# Autodesk Inventor assembly: 0005-00-03 Y axis
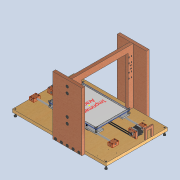
[picture p0: Inventor's stored thumbnail of the model, 180x180]
Saved by Autodesk Inventor 2020 (Build 240168000, 168)
## iProperties
Created: 2020-12-18
Part Number: 0005-00-03 Y axis
Document SubType Name: Assembly
Designer: Iulian Bors
Mass: 17144.8 g
Surface Area: 27601.7 cm^2
Volume: 16303.9 cm^3
Density: 1.05157 g/cm^3
Author: Iulian Bors
Subject: 10-03
## Documents named in this file (29)
- Z:\I.A.B\Proiecte\0005 I.A.B 3d 2.0 Imprimanta aracet\10 Mecanic\0005-10-03 Y axis.iam
- Z:\I.A.B\Proiecte\0005 I.A.B 3d 2.0 Imprimanta aracet\10 Mecanic\Foaie A4.ipt
- Z:\I.A.B\Proiecte\0005 I.A.B 3d 2.0 Imprimanta aracet\10 Mecanic\0005-10-1001 NEMA17 - Motor de passo.ipt
- Z:\I.A.B\Proiecte\0005 I.A.B 3d 2.0 Imprimanta aracet\10 Mecanic\0005-10-013 Bed.ipt
- Z:\I.A.B\Proiecte\0005 I.A.B 3d 2.0 Imprimanta aracet\10 Mecanic\0005-10-1008 Bara rectificata.ipt
- Z:\I.A.B\Proiecte\0005 I.A.B 3d 2.0 Imprimanta aracet\10 Mecanic\0005-10-014 Suport Bed.ipt
- Z:\I.A.B\Proiecte\0005 I.A.B 3d 2.0 Imprimanta aracet\10 Mecanic\0005-10-1009 LM10uu.ipt
- Z:\I.A.B\Proiecte\0005 I.A.B 3d 2.0 Imprimanta aracet\10 Mecanic\0005-10-015 suport tija.ipt
- Z:\I.A.B\Proiecte\0005 I.A.B 3d 2.0 Imprimanta aracet\10 Mecanic\0005-10-1010 GT2 Timing Pulley 20 Tooth.ipt
- Z:\I.A.B\Proiecte\0005 I.A.B 3d 2.0 Imprimanta aracet\10 Mecanic\0005-10-1011 16T W6 B3 Without T_Shrinkwrap_1.ipt
- Z:\I.A.B\Proiecte\0005 I.A.B 3d 2.0 Imprimanta aracet\10 Mecanic\0005-10-019 intinzator y.ipt
- Z:\I.A.B\Proiecte\0005 I.A.B 3d 2.0 Imprimanta aracet\10 Mecanic\0005-10-1016 curea Y.ipt
- Z:\I.A.B\Proiecte\0005 I.A.B 3d 2.0 Imprimanta aracet\10 Mecanic\0005-10-020 suport motor y.ipt
- Z:\I.A.B\Proiecte\0005 I.A.B 3d 2.0 Imprimanta aracet\10 Mecanic\0005-10-025 Activator senzor Y.ipt
- Z:\I.A.B\Proiecte\0005 I.A.B 3d 2.0 Imprimanta aracet\10 Mecanic\0005-10-1035.ipt
- Z:\I.A.B\Proiecte\0005 I.A.B 3d 2.0 Imprimanta aracet\10 Mecanic\0005-10-1036 DIN 125 - A 5.3.ipt
- Z:\I.A.B\Proiecte\0005 I.A.B 3d 2.0 Imprimanta aracet\10 Mecanic\0005-10-1037 DIN 315 - M4.ipt
- Z:\I.A.B\Proiecte\0005 I.A.B 3d 2.0 Imprimanta aracet\10 Mecanic\0005-10-1033 DIN 914 - M5 x 10.ipt
- Z:\I.A.B\Proiecte\0005 I.A.B 3d 2.0 Imprimanta aracet\10 Mecanic\0005-10-1032.ipt
- Z:\I.A.B\Proiecte\0005 I.A.B 3d 2.0 Imprimanta aracet\10 Mecanic\0005-10-1020 ISO 7089 - 3 - 140 HV(1).ipt
- Z:\I.A.B\Proiecte\0005 I.A.B 3d 2.0 Imprimanta aracet\10 Mecanic\Surub M4 saiba piulita 60mm.iam
- Z:\I.A.B\Proiecte\0005 I.A.B 3d 2.0 Imprimanta aracet\10 Mecanic\Surub M4 saiba piulita 45mm.iam
- Z:\I.A.B\Proiecte\0005 I.A.B 3d 2.0 Imprimanta aracet\10 Mecanic\0005-10-1040 Coil.iam
- Z:\I.A.B\Proiecte\0005 I.A.B 3d 2.0 Imprimanta aracet\10 Mecanic\Colier.ipt
- Z:\I.A.B\Proiecte\0005 I.A.B 3d 2.0 Imprimanta aracet\10 Mecanic\0005-10-01 Cadru_Shrinkwrap_1.ipt
- Z:\I.A.B\Proiecte\0005 I.A.B 3d 2.0 Imprimanta aracet\10 Mecanic\0005-10-1049 DIN 7991 - M4x40.ipt
- Z:\I.A.B\Proiecte\0005 I.A.B 3d 2.0 Imprimanta aracet\10 Mecanic\0005-10-1027 ISO 7050 - ST 4.2 x 32 - C - Z.ipt
- Z:\I.A.B\Proiecte\0005 I.A.B 3d 2.0 Imprimanta aracet\10 Mecanic\0005-10-1045ISO 7050 - ST 3.5 x 22 - C - Z.ipt
- Z:\I.A.B\Proiecte\0005 I.A.B 3d 2.0 Imprimanta aracet\10 Mecanic\0005-10-1051 DIN 933 - M5  x 40.ipt
## Components (80 placed, 28 different names)
1. Foaie A4.ipt:1 — Flush:29, Flush:30, Mate:47
2. 0005-10-014 Suport Bed.ipt:2 — Flush:28, Tangent:11, Tangent:12, Flush:29, Flush:30, Mate:46, Flush:32, Flush:33, Mate:48, Mate:125, Flush:67, Insert:30, Insert:31, Insert:32, Insert:33, Flush:71, Mate:132, Mate:135, Mate:136, Angle:19, Angle:20
3. 0005-10-013 Bed.ipt:7 — Mate:47, Flush:32, Flush:33, Mate:48, Insert:26, Insert:27, Insert:28, Insert:29
4. 0005-10-1001 NEMA17 - Motor de passo.ipt:8 — Mate:102, Flush:55, Flush:58
5. 0005-10-1010 GT2 Timing Pulley 20 Tooth.ipt:9 — Mate:94, Mate:95, Flush:51
6. 0005-10-1011 16T W6 B3 Without T_Shrinkwrap_1.ipt:10 — Flush:51
7. 0005-10-019 intinzator y.ipt:11 — Angle:17, Mate:128, Mate:129, Insert:22, Insert:46, Insert:47
8. 0005-10-1016 curea Y.ipt:12 — Mate:94, Mate:95, Angle:17
9. 0005-10-020 suport motor y.ipt:13 — Mate:102, Flush:55, Insert:42, Insert:43, Insert:44, Insert:45, Mate:149
10. 0005-10-025 Activator senzor Y.ipt:14 — Mate:125, Flush:67, Flush:68, Insert:52, Insert:53
11. 0005-10-01 Cadru_Shrinkwrap_1.ipt:15 — Mate:127, Flush:70, Mate:129, Angle:18, Mate:130, Insert:60, Insert:61, Insert:62, Mate:149
12. DIN 933 - M5  x 40.ipt:16 — Insert:22, Insert:23, Insert:25
13. 0005-10-1035.ipt:17 — Insert:23, Insert:24
14. 0005-10-1036 DIN 125 - A 5.3.ipt:18 — Insert:24
15. 0005-10-1036 DIN 125 - A 5.3.ipt:19 — Insert:25
16. 0005-10-1037 DIN 315 - M4.ipt:20 — Insert:26
17. 0005-10-1037 DIN 315 - M4.ipt:21 — Insert:27
18. 0005-10-1037 DIN 315 - M4.ipt:22 — Insert:28
19. 0005-10-1037 DIN 315 - M4.ipt:23 — Insert:29
20. 0005-10-1049 DIN 7991 - M4x40.ipt:24 — Insert:30, Mate:137, Mate:138
21. 0005-10-1049 DIN 7991 - M4x40.ipt:25 — Insert:31, Mate:131
22. 0005-10-1049 DIN 7991 - M4x40.ipt:26 — Insert:32, Mate:133, Mate:134
23. 0005-10-1049 DIN 7991 - M4x40.ipt:27 — Insert:33, Mate:139, Mate:140
24. 0005-10-1033 DIN 914 - M5 x 10.ipt:28 — Insert:35
25. 0005-10-1033 DIN 914 - M5 x 10.ipt:29 — Insert:54
26. 0005-10-1033 DIN 914 - M5 x 10.ipt:30 — Insert:37
27. 0005-10-1032.ipt:31
28. 0005-10-1020 ISO 7089 - 3 - 140 HV(1).ipt:32 — Insert:45
29. 0005-10-1032.ipt:33
30. 0005-10-1020 ISO 7089 - 3 - 140 HV(1).ipt:34 — Insert:44
31. 0005-10-1032.ipt:35
32. 0005-10-1020 ISO 7089 - 3 - 140 HV(1).ipt:36 — Insert:43
33. 0005-10-1032.ipt:37
34. 0005-10-1020 ISO 7089 - 3 - 140 HV(1).ipt:38 — Insert:42
35. Surub M4 saiba piulita 60mm.iam:39 [sub-assembly] — Insert:46
36. Surub M4 saiba piulita 60mm.iam:40 [sub-assembly] — Insert:47, Mate:128
37. 0005-10-1045ISO 7050 - ST 3.5 x 22 - C - Z.ipt:41 — Insert:52
38. 0005-10-1045ISO 7050 - ST 3.5 x 22 - C - Z.ipt:42 — Insert:53
39. 0005-10-1033 DIN 914 - M5 x 10.ipt:49 — Insert:55
40. 0005-10-1040 Coil.iam:66 [sub-assembly] — Mate:131, Flush:71
41. 0005-10-1040 Coil.iam:67 [sub-assembly] — Mate:132, Mate:133, Mate:134
42. 0005-10-1040 Coil.iam:68 [sub-assembly] — Mate:136, Mate:137, Mate:138
43. 0005-10-1040 Coil.iam:69 [sub-assembly] — Mate:135, Mate:139, Mate:140
44. Colier.ipt:70 — Mate:145, Flush:79, Angle:20, Flush:81, Flush:83
45. Colier.ipt:71 — Mate:144, Flush:77, Flush:78
46. Colier.ipt:72 — Mate:141, Flush:72, Angle:19, Flush:73
47. Colier.ipt:73 — Mate:143, Flush:75, Flush:76, Flush:78
48. Colier.ipt:74 — Mate:142, Flush:73, Flush:74, Flush:76
49. Colier.ipt:75 — Mate:146, Flush:80, Flush:81, Flush:85
50. Colier.ipt:76 — Mate:148, Flush:84, Flush:85
51. Colier.ipt:77 — Mate:147, Flush:82, Flush:83
52. 0005-10-1027 ISO 7050 - ST 4.2 x 32 - C - Z.ipt:78 — Insert:60
53. 0005-10-1027 ISO 7050 - ST 4.2 x 32 - C - Z.ipt:79 — Insert:61
54. 0005-10-1027 ISO 7050 - ST 4.2 x 32 - C - Z.ipt:80 — Insert:62
55. 0005-10-1009 LM10uu.ipt:3 — Flush:28, Tangent:11, Tangent:12, Mate:147, Flush:82, Mate:148, Flush:84
56. 0005-10-1009 LM10uu.ipt:4 — Mate:44, Mate:63, Mate:141, Flush:72, Mate:142, Flush:74
57. 0005-10-1009 LM10uu.ipt:5 — Flush:68, Mate:145, Flush:79, Mate:146, Flush:80
58. 0005-10-1009 LM10uu.ipt:6 — Mate:65, Mate:143, Flush:75, Mate:144, Flush:77
59. 0005-10-015 suport tija.ipt:43 — Mate:63, Flush:37, Mate:126, Mate:127, Flush:70, Insert:35, Angle:18, Insert:56
60. 0005-10-1008 Bara rectificata.ipt:44 — Mate:44, Flush:37, Mate:126, Flush:69
61. 0005-10-015 suport tija.ipt:45 — Mate:65, Flush:69, Insert:37, Mate:130, Insert:58
62. 0005-10-015 suport tija.ipt:46 — Insert:55, Insert:57
63. 0005-10-1008 Bara rectificata.ipt:47
64. 0005-10-015 suport tija.ipt:48 — Insert:54, Insert:59
65. Surub M4 saiba piulita 45mm.iam:50 [sub-assembly] — Insert:56
66. Surub M4 saiba piulita 45mm.iam:51 [sub-assembly]
67. Surub M4 saiba piulita 45mm.iam:52 [sub-assembly]
68. Surub M4 saiba piulita 45mm.iam:53 [sub-assembly]
69. Surub M4 saiba piulita 45mm.iam:54 [sub-assembly] — Insert:57
70. Surub M4 saiba piulita 45mm.iam:55 [sub-assembly]
71. Surub M4 saiba piulita 45mm.iam:56 [sub-assembly]
72. Surub M4 saiba piulita 45mm.iam:57 [sub-assembly]
73. Surub M4 saiba piulita 45mm.iam:58 [sub-assembly] — Insert:58
74. Surub M4 saiba piulita 45mm.iam:59 [sub-assembly]
75. Surub M4 saiba piulita 45mm.iam:60 [sub-assembly]
76. Surub M4 saiba piulita 45mm.iam:61 [sub-assembly]
77. Surub M4 saiba piulita 45mm.iam:62 [sub-assembly] — Insert:59
78. Surub M4 saiba piulita 45mm.iam:63 [sub-assembly]
79. Surub M4 saiba piulita 45mm.iam:64 [sub-assembly]
80. Surub M4 saiba piulita 45mm.iam:65 [sub-assembly]
## Component patterns: (4 elements, first: 0005-10-1009 LM10uu.ipt:3), (2 elements, first: 0005-10-015 suport tija.ipt:43 + 0005-10-1008 Bara rectificata.ipt:44 + 0005-10-015 suport tija.ipt:45), (4 elements, first: Surub M4 saiba piulita 45mm.iam:50), (4 elements, first: Surub M4 saiba piulita 45mm.iam:54), (4 elements, first: Surub M4 saiba piulita 45mm.iam:58), (4 elements, first: Surub M4 saiba piulita 45mm.iam:62)
## Relationships (106: Mate 36, Insert 36, Flush 28, Angle 4, Tangent 2)
- Flush:28 (75 mm): 0005-10-014 Suport Bed.ipt:2 ↔ 0005-10-1009 LM10uu.ipt:3
- Tangent:11: 0005-10-014 Suport Bed.ipt:2 ↔ 0005-10-1009 LM10uu.ipt:3
- Tangent:12 (-30 mm): 0005-10-014 Suport Bed.ipt:2 ↔ 0005-10-1009 LM10uu.ipt:3
- Mate:44: 0005-10-1009 LM10uu.ipt:4 ↔ 0005-10-1008 Bara rectificata.ipt:44
- Flush:29 (10 mm): Foaie A4.ipt:1 ↔ 0005-10-014 Suport Bed.ipt:2
- Flush:30 (12.5 mm): Foaie A4.ipt:1 ↔ 0005-10-014 Suport Bed.ipt:2
- Mate:46 (18 mm): 0005-10-014 Suport Bed.ipt:2
- Mate:47: Foaie A4.ipt:1 ↔ 0005-10-013 Bed.ipt:7
- Flush:32: 0005-10-014 Suport Bed.ipt:2 ↔ 0005-10-013 Bed.ipt:7
- Flush:33: 0005-10-014 Suport Bed.ipt:2 ↔ 0005-10-013 Bed.ipt:7
- Mate:48 (20 mm): 0005-10-014 Suport Bed.ipt:2 ↔ 0005-10-013 Bed.ipt:7
- Mate:63: 0005-10-1009 LM10uu.ipt:4 ↔ 0005-10-015 suport tija.ipt:43
- Flush:37: 0005-10-015 suport tija.ipt:43 ↔ 0005-10-1008 Bara rectificata.ipt:44
- Mate:65: 0005-10-1009 LM10uu.ipt:6 ↔ 0005-10-015 suport tija.ipt:45
- [Insert] (-13 mm): 0005-10-1001 NEMA17 - Motor de passo.ipt:8 ↔ 0005-10-1010 GT2 Timing Pulley 20 Tooth.ipt:9
- [Mate]: 0005-10-1011 16T W6 B3 Without T_Shrinkwrap_1.ipt:10 ↔ 0005-10-019 intinzator y.ipt:11
- [Mate] (1 mm): 0005-10-1011 16T W6 B3 Without T_Shrinkwrap_1.ipt:10 ↔ 0005-10-019 intinzator y.ipt:11
- Mate:94: 0005-10-1010 GT2 Timing Pulley 20 Tooth.ipt:9 ↔ 0005-10-1016 curea Y.ipt:12
- Mate:95: 0005-10-1010 GT2 Timing Pulley 20 Tooth.ipt:9 ↔ 0005-10-1016 curea Y.ipt:12
- Flush:51: 0005-10-1010 GT2 Timing Pulley 20 Tooth.ipt:9 ↔ 0005-10-1011 16T W6 B3 Without T_Shrinkwrap_1.ipt:10
- Angle:17 (0 deg): 0005-10-019 intinzator y.ipt:11 ↔ 0005-10-1016 curea Y.ipt:12
- Mate:102: 0005-10-1001 NEMA17 - Motor de passo.ipt:8 ↔ 0005-10-020 suport motor y.ipt:13
- Flush:55: 0005-10-1001 NEMA17 - Motor de passo.ipt:8 ↔ 0005-10-020 suport motor y.ipt:13
- Flush:58 (-322.09 mm): 0005-10-1001 NEMA17 - Motor de passo.ipt:8
- Mate:125: 0005-10-014 Suport Bed.ipt:2 ↔ 0005-10-025 Activator senzor Y.ipt:14
- Flush:67: 0005-10-014 Suport Bed.ipt:2 ↔ 0005-10-025 Activator senzor Y.ipt:14
- Flush:68 (-5 mm): 0005-10-025 Activator senzor Y.ipt:14 ↔ 0005-10-1009 LM10uu.ipt:5
- Mate:126: 0005-10-015 suport tija.ipt:43 ↔ 0005-10-1008 Bara rectificata.ipt:44
- Flush:69: 0005-10-1008 Bara rectificata.ipt:44 ↔ 0005-10-015 suport tija.ipt:45
- Mate:127: 0005-10-01 Cadru_Shrinkwrap_1.ipt:15 ↔ 0005-10-015 suport tija.ipt:43
- Flush:70 (5 mm): 0005-10-01 Cadru_Shrinkwrap_1.ipt:15 ↔ 0005-10-015 suport tija.ipt:43
- Mate:128: 0005-10-019 intinzator y.ipt:11 ↔ Surub M4 saiba piulita 60mm.iam:40
- Mate:129: 0005-10-019 intinzator y.ipt:11 ↔ 0005-10-01 Cadru_Shrinkwrap_1.ipt:15
- Insert:22 (1.2 mm): 0005-10-019 intinzator y.ipt:11 ↔ DIN 933 - M5  x 40.ipt:16
- Insert:23 (5 mm): DIN 933 - M5  x 40.ipt:16 ↔ 0005-10-1035.ipt:17
- Insert:24: 0005-10-1035.ipt:17 ↔ 0005-10-1036 DIN 125 - A 5.3.ipt:18
- Insert:25: DIN 933 - M5  x 40.ipt:16 ↔ 0005-10-1036 DIN 125 - A 5.3.ipt:19
- Insert:26: 0005-10-013 Bed.ipt:7 ↔ 0005-10-1037 DIN 315 - M4.ipt:20
- Insert:27: 0005-10-013 Bed.ipt:7 ↔ 0005-10-1037 DIN 315 - M4.ipt:21
- Insert:28: 0005-10-013 Bed.ipt:7 ↔ 0005-10-1037 DIN 315 - M4.ipt:22
- Insert:29: 0005-10-013 Bed.ipt:7 ↔ 0005-10-1037 DIN 315 - M4.ipt:23
- Insert:30: 0005-10-014 Suport Bed.ipt:2 ↔ 0005-10-1049 DIN 7991 - M4x40.ipt:24
- Insert:31: 0005-10-014 Suport Bed.ipt:2 ↔ 0005-10-1049 DIN 7991 - M4x40.ipt:25
- Insert:32: 0005-10-014 Suport Bed.ipt:2 ↔ 0005-10-1049 DIN 7991 - M4x40.ipt:26
- Insert:33: 0005-10-014 Suport Bed.ipt:2 ↔ 0005-10-1049 DIN 7991 - M4x40.ipt:27
- Insert:35: 0005-10-1033 DIN 914 - M5 x 10.ipt:28 ↔ 0005-10-015 suport tija.ipt:43
- Insert:37: 0005-10-1033 DIN 914 - M5 x 10.ipt:30 ↔ 0005-10-015 suport tija.ipt:45
- [Insert]: 0005-10-1032.ipt:31 ↔ 0005-10-1020 ISO 7089 - 3 - 140 HV(1).ipt:32
- [Insert]: 0005-10-1032.ipt:33 ↔ 0005-10-1020 ISO 7089 - 3 - 140 HV(1).ipt:34
- [Insert]: 0005-10-1032.ipt:35 ↔ 0005-10-1020 ISO 7089 - 3 - 140 HV(1).ipt:36
- [Insert]: 0005-10-1032.ipt:37 ↔ 0005-10-1020 ISO 7089 - 3 - 140 HV(1).ipt:38
- Insert:42: 0005-10-020 suport motor y.ipt:13 ↔ 0005-10-1020 ISO 7089 - 3 - 140 HV(1).ipt:38
- Insert:43: 0005-10-020 suport motor y.ipt:13 ↔ 0005-10-1020 ISO 7089 - 3 - 140 HV(1).ipt:36
- Insert:44: 0005-10-020 suport motor y.ipt:13 ↔ 0005-10-1020 ISO 7089 - 3 - 140 HV(1).ipt:34
- Insert:45: 0005-10-020 suport motor y.ipt:13 ↔ 0005-10-1020 ISO 7089 - 3 - 140 HV(1).ipt:32
- Insert:46: 0005-10-019 intinzator y.ipt:11 ↔ Surub M4 saiba piulita 60mm.iam:39
- Insert:47: 0005-10-019 intinzator y.ipt:11 ↔ Surub M4 saiba piulita 60mm.iam:40
- Insert:52: 0005-10-025 Activator senzor Y.ipt:14 ↔ 0005-10-1045ISO 7050 - ST 3.5 x 22 - C - Z.ipt:41
- Insert:53: 0005-10-025 Activator senzor Y.ipt:14 ↔ 0005-10-1045ISO 7050 - ST 3.5 x 22 - C - Z.ipt:42
- Angle:18 (0 deg): 0005-10-01 Cadru_Shrinkwrap_1.ipt:15 ↔ 0005-10-015 suport tija.ipt:43
- Mate:130: 0005-10-01 Cadru_Shrinkwrap_1.ipt:15 ↔ 0005-10-015 suport tija.ipt:45
- Insert:54: 0005-10-1033 DIN 914 - M5 x 10.ipt:29 ↔ 0005-10-015 suport tija.ipt:48
- Insert:55: 0005-10-1033 DIN 914 - M5 x 10.ipt:49 ↔ 0005-10-015 suport tija.ipt:46
- Insert:56: 0005-10-015 suport tija.ipt:43 ↔ Surub M4 saiba piulita 45mm.iam:50
- Insert:57: 0005-10-015 suport tija.ipt:46 ↔ Surub M4 saiba piulita 45mm.iam:54
- Insert:58: 0005-10-015 suport tija.ipt:45 ↔ Surub M4 saiba piulita 45mm.iam:58
- Insert:59: 0005-10-015 suport tija.ipt:48 ↔ Surub M4 saiba piulita 45mm.iam:62
- Mate:131: 0005-10-1049 DIN 7991 - M4x40.ipt:25 ↔ 0005-10-1040 Coil.iam:66
- Flush:71: 0005-10-014 Suport Bed.ipt:2 ↔ 0005-10-1040 Coil.iam:66
- Mate:132: 0005-10-014 Suport Bed.ipt:2 ↔ 0005-10-1040 Coil.iam:67
- Mate:133: 0005-10-1049 DIN 7991 - M4x40.ipt:26 ↔ 0005-10-1040 Coil.iam:67
- Mate:134: 0005-10-1049 DIN 7991 - M4x40.ipt:26 ↔ 0005-10-1040 Coil.iam:67
- Mate:135: 0005-10-014 Suport Bed.ipt:2 ↔ 0005-10-1040 Coil.iam:69
- Mate:136: 0005-10-014 Suport Bed.ipt:2 ↔ 0005-10-1040 Coil.iam:68
- Mate:137: 0005-10-1049 DIN 7991 - M4x40.ipt:24 ↔ 0005-10-1040 Coil.iam:68
- Mate:138: 0005-10-1049 DIN 7991 - M4x40.ipt:24 ↔ 0005-10-1040 Coil.iam:68
- Mate:139: 0005-10-1049 DIN 7991 - M4x40.ipt:27 ↔ 0005-10-1040 Coil.iam:69
- Mate:140: 0005-10-1049 DIN 7991 - M4x40.ipt:27 ↔ 0005-10-1040 Coil.iam:69
- Mate:141: Colier.ipt:72 ↔ 0005-10-1009 LM10uu.ipt:4
- Flush:72: Colier.ipt:72 ↔ 0005-10-1009 LM10uu.ipt:4
- Angle:19 (0 deg): 0005-10-014 Suport Bed.ipt:2 ↔ Colier.ipt:72
- Mate:142: Colier.ipt:74 ↔ 0005-10-1009 LM10uu.ipt:4
- Flush:73: Colier.ipt:72 ↔ Colier.ipt:74
- Flush:74: Colier.ipt:74 ↔ 0005-10-1009 LM10uu.ipt:4
- Mate:143: Colier.ipt:73 ↔ 0005-10-1009 LM10uu.ipt:6
- Flush:75: Colier.ipt:73 ↔ 0005-10-1009 LM10uu.ipt:6
- Flush:76: Colier.ipt:73 ↔ Colier.ipt:74
- Mate:144: Colier.ipt:71 ↔ 0005-10-1009 LM10uu.ipt:6
- Flush:77: Colier.ipt:71 ↔ 0005-10-1009 LM10uu.ipt:6
- Flush:78: Colier.ipt:71 ↔ Colier.ipt:73
- Mate:145: Colier.ipt:70 ↔ 0005-10-1009 LM10uu.ipt:5
- Flush:79: Colier.ipt:70 ↔ 0005-10-1009 LM10uu.ipt:5
- Angle:20 (0 deg): 0005-10-014 Suport Bed.ipt:2 ↔ Colier.ipt:70
- Mate:146: Colier.ipt:75 ↔ 0005-10-1009 LM10uu.ipt:5
- Flush:80: Colier.ipt:75 ↔ 0005-10-1009 LM10uu.ipt:5
- Flush:81: Colier.ipt:70 ↔ Colier.ipt:75
- Mate:147: Colier.ipt:77 ↔ 0005-10-1009 LM10uu.ipt:3
- Flush:82: Colier.ipt:77 ↔ 0005-10-1009 LM10uu.ipt:3
- Flush:83: Colier.ipt:70 ↔ Colier.ipt:77
- Mate:148: Colier.ipt:76 ↔ 0005-10-1009 LM10uu.ipt:3
- Flush:84: Colier.ipt:76 ↔ 0005-10-1009 LM10uu.ipt:3
- Flush:85: Colier.ipt:75 ↔ Colier.ipt:76
- Insert:60: 0005-10-01 Cadru_Shrinkwrap_1.ipt:15 ↔ 0005-10-1027 ISO 7050 - ST 4.2 x 32 - C - Z.ipt:78
- Insert:61: 0005-10-01 Cadru_Shrinkwrap_1.ipt:15 ↔ 0005-10-1027 ISO 7050 - ST 4.2 x 32 - C - Z.ipt:79
- Insert:62: 0005-10-01 Cadru_Shrinkwrap_1.ipt:15 ↔ 0005-10-1027 ISO 7050 - ST 4.2 x 32 - C - Z.ipt:80
- Mate:149: 0005-10-020 suport motor y.ipt:13 ↔ 0005-10-01 Cadru_Shrinkwrap_1.ipt:15
## Named parameters: d217_d198 = -13 mm, d221_d205 = 1 mm, d222_d204 = 0 mm, d391_d441 = 0 mm, d392_d441 = 0 mm, d393_d441 = 0 mm
